# Autodesk Inventor assembly: TL20240701-10100CV-PROFILE
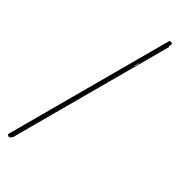
[picture p0: Inventor's stored thumbnail of the model, 180x180]
Saved by Autodesk Inventor 2022.5 (Build 265521000, 521)
## iProperties
Category: CONVEYOR ASSY
Company: 현대트랜시스(대유)
Created: 2023-04-05
Part Number: TL20240701-10100CV-PROFILE
Description: 0
Document SubType Name: Assembly
Designer: 박성규
User Status: 1 x48
Stock Number: 000
Project: SW-PJT
Checked By: 김형민
Engr Approved By: 김시현
Mfg Approved By: 호상태
Mass: 272676 g
Surface Area: 166429 cm^2
Volume: 36646.5 cm^3
Density: 7.44071 g/cm^3
DocNumber: TN20221101-FA000000-000-1.iam
Folder: OLD\개발설비\1. 사내개발\19. 미쓰비시 컨버팅 솔루션 데모장비\
Detail Description: Processed products
Title: PROFILE
Subject: SW차종 시트조립라인
Author: 박성규
Revision Number: A
## Documents named in this file (11)
- D:\V\Designs\프로젝트 자산\자동화 & 스마트팩토리\현대트랜시스(구 다이모스, 파워텍)\현대트랜시스(대유화성공장)_SW 시트조립라인\2.제작도면\1. 1ST LINE\CONVEYOR\TL20240701-10100CV\TL20240701-10100CV-PROFILE ASSY.iam
- D:\V\Designs\프로젝트 자산\자동화 & 스마트팩토리\현대트랜시스(구 다이모스, 파워텍)\현대트랜시스(대유화성공장)_SW 시트조립라인\2.제작도면\1. 1ST LINE\CONVEYOR\TL20240701-10100CV\TL20240701-10100CV-DY1055.ipt
- D:\V\Designs\프로젝트 자산\자동화 & 스마트팩토리\현대트랜시스(구 다이모스, 파워텍)\현대트랜시스(대유화성공장)_SW 시트조립라인\2.제작도면\1. 1ST LINE\CONVEYOR\TL20240701-10100CV\TL20240701-10100CV-GUIDE RAIL_H-21.ipt
- D:\V\Designs\프로젝트 자산\자동화 & 스마트팩토리\현대트랜시스(구 다이모스, 파워텍)\현대트랜시스(대유화성공장)_SW 시트조립라인\2.제작도면\1. 1ST LINE\CONVEYOR\TL20240701-10100CV\TL20240701-10100CV-RAIL 1.ipt
- D:\V\Designs\프로젝트 자산\자동화 & 스마트팩토리\현대트랜시스(구 다이모스, 파워텍)\현대트랜시스(대유화성공장)_SW 시트조립라인\2.제작도면\1. 1ST LINE\CONVEYOR\TL20240701-10100CV\TL20240701-10100CV-RAIL 2.ipt
- D:\V\Designs\프로젝트 자산\자동화 & 스마트팩토리\현대트랜시스(구 다이모스, 파워텍)\현대트랜시스(대유화성공장)_SW 시트조립라인\2.제작도면\1. 1ST LINE\CONVEYOR\TL20240701-10100CV\TL20240701-10100CV-DY1054-1.ipt
- D:\V\Designs\프로젝트 자산\자동화 & 스마트팩토리\현대트랜시스(구 다이모스, 파워텍)\현대트랜시스(대유화성공장)_SW 시트조립라인\2.제작도면\1. 1ST LINE\CONVEYOR\TL20240701-10100CV\TL20240701-10100CV-DY1054-2.ipt
- D:\V\Designs\프로젝트 자산\자동화 & 스마트팩토리\현대트랜시스(구 다이모스, 파워텍)\현대트랜시스(대유화성공장)_SW 시트조립라인\2.제작도면\1. 1ST LINE\CONVEYOR\TL20240701-10100CV\TL20240701-10100CV-001.ipt
- D:\V\Designs\프로젝트 자산\자동화 & 스마트팩토리\현대트랜시스(구 다이모스, 파워텍)\현대트랜시스(대유화성공장)_SW 시트조립라인\2.제작도면\1. 1ST LINE\CONVEYOR\TL20240701-10100CV\TL20240701-10100CV-002.ipt
- D:\V\Designs\프로젝트 자산\자동화 & 스마트팩토리\현대트랜시스(구 다이모스, 파워텍)\현대트랜시스(대유화성공장)_SW 시트조립라인\2.제작도면\1. 1ST LINE\CONVEYOR\TL20240701-10100CV\TL20240701-10100CV-003.ipt
- D:\V\Designs\프로젝트 자산\자동화 & 스마트팩토리\현대트랜시스(구 다이모스, 파워텍)\현대트랜시스(대유화성공장)_SW 시트조립라인\2.제작도면\1. 1ST LINE\CONVEYOR\TL20240701-10100CV\TL20240701-10100CV-004.ipt
## Components (16 placed, 10 different names)
1. TL20240701-10100CV-RAIL 2.ipt:1 — 메이트:9, 메이트:10, Flush:40
2. TL20240701-10100CV-DY1054-1.ipt:1 — 메이트:1, 메이트:2, 플러쉬:1, 메이트:4, 메이트:5, 메이트:6, 플러쉬:6, 메이트:7, 메이트:8, 메이트:9, 메이트:10, 메이트:19, 플러쉬:21, 플러쉬:22, Mate:20, Flush:25, Flush:26, Mate:34, Mate:36, Mate:39, Mate:41, Mate:42, Flush:37, Flush:38, Flush:39, Mate:44, Flush:41, Flush:42
3. TL20240701-10100CV-DY1055.ipt:1 — 메이트:6, 플러쉬:6, Flush:37
4. TL20240701-10100CV-DY1055.ipt:2 — 메이트:7, 메이트:8, Flush:38
5. TL20240701-10100CV-GUIDE RAIL_H-21.ipt:1 — 메이트:4, 메이트:5, Flush:39
6. TL20240701-10100CV-RAIL 1.ipt:1 — 메이트:19, 플러쉬:21, 플러쉬:22
7. TL20240701-10100CV-RAIL 1.ipt:2 — Mate:44, Flush:41, Flush:42
8. TL20240701-10100CV-DY1054-2.ipt:1 — Mate:20, Flush:25, Flush:26, Mate:35, Mate:37, Mate:38, Mate:40, Mate:43, Flush:36, Flush:40
9. TL20240701-10100CV-001.ipt:1 — Mate:36, Mate:37
10. TL20240701-10100CV-002.ipt:1 — Mate:38, Mate:39, Mate:42, Mate:43
11. TL20240701-10100CV-001.ipt:2 — Mate:34, Mate:35, Mate:40, Mate:41, Flush:36
12. TL20240701-10100CV-003.ipt:1
13. TL20240701-10100CV-003.ipt:2
14. TL20240701-10100CV-003.ipt:3
15. TL20240701-10100CV-003.ipt:4
16. TL20240701-10100CV-004.ipt:1
## Relationships (57: Mate 35, Flush 22)
- 메이트:1 [Mate]: TL20240701-10100CV-DY1054-1.ipt:1
- 메이트:2 [Mate]: TL20240701-10100CV-DY1054-1.ipt:1
- 플러쉬:1 [Flush]: TL20240701-10100CV-DY1054-1.ipt:1
- 메이트:4 [Mate]: TL20240701-10100CV-DY1054-1.ipt:1 ↔ TL20240701-10100CV-GUIDE RAIL_H-21.ipt:1
- 메이트:5 [Mate]: TL20240701-10100CV-DY1054-1.ipt:1 ↔ TL20240701-10100CV-GUIDE RAIL_H-21.ipt:1
- 메이트:6 [Mate]: TL20240701-10100CV-DY1054-1.ipt:1 ↔ TL20240701-10100CV-DY1055.ipt:1
- 플러쉬:6 [Flush]: TL20240701-10100CV-DY1054-1.ipt:1 ↔ TL20240701-10100CV-DY1055.ipt:1
- 메이트:7 [Mate]: TL20240701-10100CV-DY1054-1.ipt:1 ↔ TL20240701-10100CV-DY1055.ipt:2
- 메이트:8 [Mate] (0.2 mm): TL20240701-10100CV-DY1054-1.ipt:1 ↔ TL20240701-10100CV-DY1055.ipt:2
- 메이트:9 [Mate]: TL20240701-10100CV-RAIL 2.ipt:1 ↔ TL20240701-10100CV-DY1054-1.ipt:1
- 메이트:10 [Mate] (0.25 mm): TL20240701-10100CV-RAIL 2.ipt:1 ↔ TL20240701-10100CV-DY1054-1.ipt:1
- 메이트:19 [Mate]: TL20240701-10100CV-DY1054-1.ipt:1 ↔ TL20240701-10100CV-RAIL 1.ipt:1
- 플러쉬:21 [Flush]: TL20240701-10100CV-DY1054-1.ipt:1 ↔ TL20240701-10100CV-RAIL 1.ipt:1
- 플러쉬:22 [Flush]: TL20240701-10100CV-DY1054-1.ipt:1 ↔ TL20240701-10100CV-RAIL 1.ipt:1
- Mate:20: TL20240701-10100CV-DY1054-1.ipt:1 ↔ TL20240701-10100CV-DY1054-2.ipt:1
- Flush:25: TL20240701-10100CV-DY1054-1.ipt:1 ↔ TL20240701-10100CV-DY1054-2.ipt:1
- Flush:26: TL20240701-10100CV-DY1054-1.ipt:1 ↔ TL20240701-10100CV-DY1054-2.ipt:1
- [Flush]: TL20240701-10100CV-001.ipt:1 ↔ TL20240701-10100CV-002.ipt:1
- [Flush]: TL20240701-10100CV-001.ipt:1 ↔ TL20240701-10100CV-001.ipt:2
- [Flush]: TL20240701-10100CV-001.ipt:1 ↔ TL20240701-10100CV-001.ipt:2
- [Flush]: TL20240701-10100CV-001.ipt:2 ↔ TL20240701-10100CV-003.ipt:1
- [Mate]: TL20240701-10100CV-001.ipt:2 ↔ TL20240701-10100CV-003.ipt:1
- [Mate]: TL20240701-10100CV-001.ipt:2 ↔ TL20240701-10100CV-003.ipt:1
- [Mate] (5 mm): TL20240701-10100CV-001.ipt:2 ↔ TL20240701-10100CV-003.ipt:1
- [Mate]: TL20240701-10100CV-001.ipt:2 ↔ TL20240701-10100CV-003.ipt:2
- [Mate]: TL20240701-10100CV-001.ipt:2 ↔ TL20240701-10100CV-003.ipt:2
- [Flush]: TL20240701-10100CV-003.ipt:1 ↔ TL20240701-10100CV-003.ipt:2
- [Flush]: TL20240701-10100CV-003.ipt:1 ↔ TL20240701-10100CV-003.ipt:2
- [Flush]: TL20240701-10100CV-003.ipt:1 ↔ TL20240701-10100CV-003.ipt:3
- [Mate]: TL20240701-10100CV-001.ipt:1 ↔ TL20240701-10100CV-003.ipt:3
- [Mate]: TL20240701-10100CV-001.ipt:1 ↔ TL20240701-10100CV-003.ipt:3
- [Mate] (5 mm): TL20240701-10100CV-001.ipt:1 ↔ TL20240701-10100CV-003.ipt:3
- [Flush]: TL20240701-10100CV-003.ipt:2 ↔ TL20240701-10100CV-003.ipt:4
- [Mate]: TL20240701-10100CV-001.ipt:1 ↔ TL20240701-10100CV-003.ipt:4
- [Mate]: TL20240701-10100CV-001.ipt:1 ↔ TL20240701-10100CV-003.ipt:4
- [Flush]: TL20240701-10100CV-003.ipt:3 ↔ TL20240701-10100CV-003.ipt:4
- [Mate]: TL20240701-10100CV-002.ipt:1 ↔ TL20240701-10100CV-004.ipt:1
- [Mate]: TL20240701-10100CV-002.ipt:1 ↔ TL20240701-10100CV-004.ipt:1
- [Mate] (5 mm): TL20240701-10100CV-002.ipt:1 ↔ TL20240701-10100CV-004.ipt:1
- Mate:34: TL20240701-10100CV-DY1054-1.ipt:1 ↔ TL20240701-10100CV-001.ipt:2
- Mate:35: TL20240701-10100CV-DY1054-2.ipt:1 ↔ TL20240701-10100CV-001.ipt:2
- Mate:36: TL20240701-10100CV-DY1054-1.ipt:1 ↔ TL20240701-10100CV-001.ipt:1
- Mate:37: TL20240701-10100CV-DY1054-2.ipt:1 ↔ TL20240701-10100CV-001.ipt:1
- Mate:38: TL20240701-10100CV-DY1054-2.ipt:1 ↔ TL20240701-10100CV-002.ipt:1
- Mate:39: TL20240701-10100CV-DY1054-1.ipt:1 ↔ TL20240701-10100CV-002.ipt:1
- Mate:40 (3.5 mm): TL20240701-10100CV-DY1054-2.ipt:1 ↔ TL20240701-10100CV-001.ipt:2
- Mate:41 (3.5 mm): TL20240701-10100CV-DY1054-1.ipt:1 ↔ TL20240701-10100CV-001.ipt:2
- Mate:42 (4.25 mm): TL20240701-10100CV-DY1054-1.ipt:1 ↔ TL20240701-10100CV-002.ipt:1
- Mate:43 (4.25 mm): TL20240701-10100CV-DY1054-2.ipt:1 ↔ TL20240701-10100CV-002.ipt:1
- Flush:36: TL20240701-10100CV-DY1054-2.ipt:1 ↔ TL20240701-10100CV-001.ipt:2
- Flush:37: TL20240701-10100CV-DY1054-1.ipt:1 ↔ TL20240701-10100CV-DY1055.ipt:1
- Flush:38: TL20240701-10100CV-DY1054-1.ipt:1 ↔ TL20240701-10100CV-DY1055.ipt:2
- Flush:39: TL20240701-10100CV-DY1054-1.ipt:1 ↔ TL20240701-10100CV-GUIDE RAIL_H-21.ipt:1
- Flush:40: TL20240701-10100CV-RAIL 2.ipt:1 ↔ TL20240701-10100CV-DY1054-2.ipt:1
- Mate:44: TL20240701-10100CV-DY1054-1.ipt:1 ↔ TL20240701-10100CV-RAIL 1.ipt:2
- Flush:41: TL20240701-10100CV-DY1054-1.ipt:1 ↔ TL20240701-10100CV-RAIL 1.ipt:2
- Flush:42: TL20240701-10100CV-DY1054-1.ipt:1 ↔ TL20240701-10100CV-RAIL 1.ipt:2
